# Autodesk Inventor assembly: USB4105-15-A
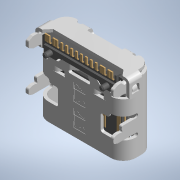
[picture p0: Inventor's stored thumbnail of the model, 180x180]
Saved by Autodesk Inventor 2020.1 (Build 241239000, 239)
## iProperties
Part Number: USB4105-15-A
Catalog Web Link: www.cadenas.de
Description: USB4105-
Vendor: GCT
Document SubType Name: Assembly
Designer: partserver
Manufacturer: GCT
Mass: 0.1332 g
Surface Area: 7.20421 cm^2
Volume: 0.1332 cm^3
Density: 1 g/cm^3
Category: PARTsolutions
Company: GCT
PSOL_IDENT_0: {$CADENAS_DATA\23d-libs\gct\usb_connector\type_c\type_c\horizontal\usb4105\usb4105.prj},176 {STYP=AS
PSOL_IDENT_1: S},{VTYP=3D},{NB=USB4105-15-A},{LINA=USB4105-15-A},{NN=USB4105},{DATE=06.12.2019 14:21:47},{GEOMDATE=
PSOL_IDENT_2: 03.12.2019 09:52:34},{VERSION=},{LINEID=10},{WBVAR=},{WBNUMERIC=}  {NB=USB4105-15-A},{LINA=USB4105-1
PSOL_IDENT_3: 5-A},{KT=DUMMY},{SHA256=LJbv6moXW0rG8uRbobPgZaOAea5zNgrCO4JnRlymaO0=},{INAME=3dmodel_usb4105_15_a_re
PSOL_IDENT_4: va1},{NAME=3dmodel_usb4105_15_a_reva1},{WEB=https://gct.co/connector/USB4105},{OC=USB4105-15-A},{PLA
PSOL_IDENT_5: TING=15 = 15μ\" Gold},{PACK=A = Tape and Reel},{REV=A1},{REVDAT=14.10.2019},{DISCLAIMER=The creation
PSOL_IDENT_6: and usage of 3D models generated by this builder are covered in our disclaimer which can be viewed
PSOL_IDENT_7: here}
NB: USB4105-15-A
NN: USB4105
NBSYN: $OC.
LINA: USB4105-15-A
CATALOG: Global Connector Technology
WEB: https://gct.co/connector/USB4105
OC: USB4105-15-A
PLATING: 15 = 15μ" Gold
PACK: A = Tape and Reel
REV: A1
REVDAT: 14.10.2019
DISCLAIMER: The creation and usage of 3D models generated by this builder are covered in our disclaimer which can be viewed here
SUPPLIER: GCT
ARTICLENO: USB4105-15-A
BOMINFO: USB4105-15-A
CREATOR: CADENAS GmbH
Title: USB4105-15-A
Author: Cadenas PARTsolutions
## Documents named in this file (3)
- C:\Users\Public\Documents\Altium\AD20\Library\libysk\3D Models\GCT\USB4105-15-A.iam
- C:\Users\Public\Documents\Altium\AD20\Library\libysk\3D Models\GCT\USB4105-15-A_PART1.ipt
- C:\Users\Public\Documents\Altium\AD20\Library\libysk\3D Models\GCT\USB4105-15-A_PART2.ipt
## Components (2 placed, 2 different names)
1. USB4105-15-A_PART1:1 — Flush:1, Flush:2, Flush:3, Mate:1, Flush:4, Flush:5
2. USB4105-15-A_PART2:1 — Flush:1, Flush:2, Flush:3
## Relationships (6: Flush 5, Mate 1)
- Flush:1: USB4105-15-A_PART1:1 ↔ USB4105-15-A_PART2:1
- Flush:2: USB4105-15-A_PART1:1 ↔ USB4105-15-A_PART2:1
- Flush:3: USB4105-15-A_PART1:1 ↔ USB4105-15-A_PART2:1
- Mate:1: USB4105-15-A_PART1:1
- Flush:4: USB4105-15-A_PART1:1
- Flush:5 (-4.47 mm): USB4105-15-A_PART1:1
